# Autodesk Inventor assembly: Ice Cream Assembly
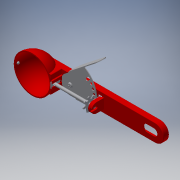
[picture p0: Inventor's stored thumbnail of the model, 180x180]
Saved by Autodesk Inventor 2016 (Build 200138000, 138)
## iProperties
Created: 2016-11-09
Part Number: Ice Cream Assembly
Document SubType Name: Assembly
Designer: Muhammad
Author: Muhammad
## Documents named in this file (7)
- C:\Users\Muhammad\Desktop\Icecream scoop\Ice Cream Assembly.iam
- C:\Users\Muhammad\Desktop\Icecream scoop\Scoop.ipt
- C:\Users\Muhammad\Desktop\Icecream scoop\Rectangular Piece.ipt
- C:\Users\Muhammad\Desktop\Icecream scoop\Thumb plate.ipt
- C:\Users\Muhammad\Desktop\Icecream scoop\Screw.ipt
- C:\Users\Muhammad\Desktop\Icecream scoop\Circular Module.ipt
- C:\Users\Muhammad\Desktop\Icecream scoop\Main turning shaft.ipt
## Components (6 placed, 6 different names)
1. Scoop:1 — Insert:1, Insert:2, Insert:3, Insert:4, Mate:1
2. Rectangular Piece:1 — Insert:1
3. Thumb plate:1 — Insert:2
4. Screw:1 — Insert:3
5. Circular Module:1 — Mate:1
6. Main turning shaft:1 — Insert:4
## Relationships (5: Insert 4, Mate 1)
- Insert:1: Scoop:1 ↔ Rectangular Piece:1
- Insert:2: Scoop:1 ↔ Thumb plate:1
- Insert:3: Scoop:1 ↔ Screw:1
- Insert:4: Scoop:1 ↔ Main turning shaft:1
- Mate:1: Scoop:1 ↔ Circular Module:1
